# Autodesk Inventor assembly: 20kg Servo
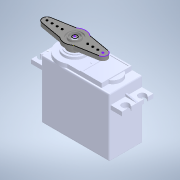
[picture p0: Inventor's stored thumbnail of the model, 180x180]
Saved by Autodesk Inventor 2020 (Build 240168000, 168)
## iProperties
Created: 2020-04-13
Part Number: 20kg Servo
Document SubType Name: Assembly
Designer: varun
Author: varun
## Documents named in this file (3)
- C:\Users\varun\Desktop\ServoArm\20kg Servo.iam
- C:\Users\varun\Desktop\ServoArm\Large Servo.ipt
- C:\Users\varun\Desktop\ServoArm\TOWER PRO MG-995, ANALOG SERVO, HORN.ipt
## Components (2 placed, 2 different names)
1. Large Servo:1 — Mate:1, Mate:2, Angle:1
2. TOWER PRO MG-995, ANALOG SERVO, HORN:1 — Mate:1, Mate:2, Angle:1
## Relationships (3: Mate 2, Angle 1)
- Mate:1: Large Servo:1 ↔ TOWER PRO MG-995, ANALOG SERVO, HORN:1
- Mate:2: Large Servo:1 ↔ TOWER PRO MG-995, ANALOG SERVO, HORN:1
- Angle:1 (0 deg): Large Servo:1 ↔ TOWER PRO MG-995, ANALOG SERVO, HORN:1
